# Autodesk Inventor assembly: DoorLockAssembly
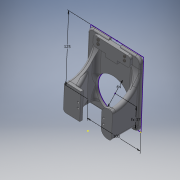
[picture p0: Inventor's stored thumbnail of the model, 180x180]
Saved by Autodesk Inventor 2019 (Build 230136000, 136)
## iProperties
Created: 2019-05-08
Part Number: DoorLockAssembly
Document SubType Name: Assembly
Designer: Iván
Author: Iván
## Documents named in this file (7)
- C:\Users\Iván\Documents\Github\DoorLock\LockSupport\DoorLockAssembly.iam
- C:\Users\Iván\Documents\Github\DoorLock\LockSupport\RotationLock.ipt
- C:\Users\Iván\Documents\Github\DoorLock\LockSupport\DoorLockSupport.ipt
- C:\Users\Iván\Documents\Github\DoorLock\LockSupport\DoorLockAssembly\Design Accelerator\Bolted Connection1.iam
- C:\Users\Iván\Documents\Github\DoorLock\LockSupport\DoorLockAssembly\Design Accelerator\Bolted Connection3.iam
- C:\Users\Iván\Documents\Github\DoorLock\LockSupport\DoorLockAssembly\Design Accelerator\Bolted Connection4.iam
- C:\Users\Iván\Documents\Github\DoorLock\LockSupport\DoorLockAssembly\Design Accelerator\Bolted Connection6.iam
## Components (6 placed, 3 different names)
1. DoorLockSupport:1 — Mate:1, Mate:2, Mate:3, Mate:10, Mate:12, Mate:13, Mate:14, Mate:15, Mate:16, Mate:17
2. RotationLock:1 — Mate:1, Mate:2, Mate:3, Mate:11
3. Bolted Connection:1 [sub-assembly] — Mate:10, Mate:11
4. Bolted Connection:2 [sub-assembly] — Mate:12, Mate:13
5. Bolted Connection:3 [sub-assembly] — Mate:14, Mate:15
6. Bolted Connection:4 [sub-assembly] — Mate:16, Mate:17
## Relationships (11: Mate 11)
- Mate:1: DoorLockSupport:1 ↔ RotationLock:1
- Mate:2: DoorLockSupport:1 ↔ RotationLock:1
- Mate:3: DoorLockSupport:1 ↔ RotationLock:1
- Mate:10: DoorLockSupport:1 ↔ Bolted Connection:1
- Mate:11: RotationLock:1 ↔ Bolted Connection:1
- Mate:12: DoorLockSupport:1 ↔ Bolted Connection:2
- Mate:13: DoorLockSupport:1 ↔ Bolted Connection:2
- Mate:14: DoorLockSupport:1 ↔ Bolted Connection:3
- Mate:15: DoorLockSupport:1 ↔ Bolted Connection:3
- Mate:16: DoorLockSupport:1 ↔ Bolted Connection:4
- Mate:17: DoorLockSupport:1 ↔ Bolted Connection:4
